# Autodesk Inventor assembly: E3D-HotEnd
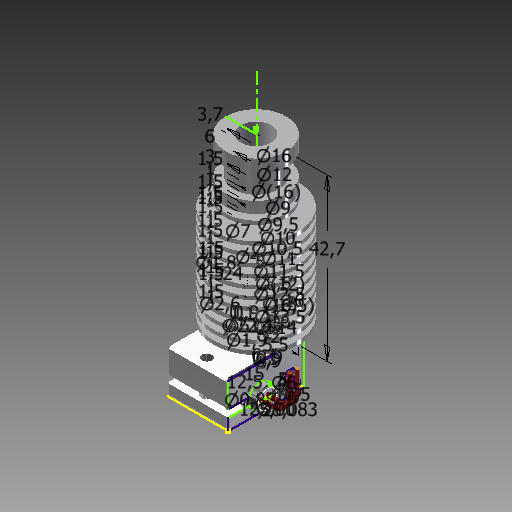
[picture p0: Inventor's stored thumbnail of the model, 512x512]
Saved by Autodesk Inventor 2018 (Build 220112000, 112)
## iProperties
Created: 2015-02-05
Part Number: E3D-HotEnd
Document SubType Name: Assembly
Designer: Parabolik
Author: Parabolik
## Documents named in this file (6)
- C:\Users\Till\Dropbox\DIY\CoreBot\CAD Parts\E3D-HotEnd\E3D-HotEnd.iam
- C:\Users\Till\Dropbox\DIY\CoreBot\CAD Parts\E3D-HotEnd\heater.ipt
- C:\Users\Till\Dropbox\DIY\CoreBot\CAD Parts\E3D-HotEnd\heater-cartrig.ipt
- C:\Users\Till\Dropbox\DIY\CoreBot\CAD Parts\E3D-HotEnd\nozzls\nozzle-0,4.ipt
- C:\Users\Till\Dropbox\DIY\CoreBot\CAD Parts\E3D-HotEnd\Heat Break.ipt
- C:\Users\Till\Dropbox\DIY\CoreBot\CAD Parts\E3D-HotEnd\HeatSink.ipt
## Components (5 placed, 5 different names)
1. heater:1 — Жесткий:3, Жесткий:8, Жесткий:7
2. heater-cartrig:1 — Жесткий:3
3. nozzle-0,4:1 — Жесткий:7
4. Heat Break:1 — Жесткий:6, Жесткий:8
5. HeatSink:1 — Жесткий:6
## Relationships (4: WeldJoint 4)
- Жесткий:3 [WeldJoint]: heater:1 ↔ heater-cartrig:1
- Жесткий:6 [WeldJoint]: Heat Break:1 ↔ HeatSink:1
- Жесткий:8 [WeldJoint]: heater:1 ↔ Heat Break:1
- Жесткий:7 [WeldJoint] (0.1 mm): heater:1 ↔ nozzle-0,4:1
